# Autodesk Inventor assembly: IDLE ROLLER
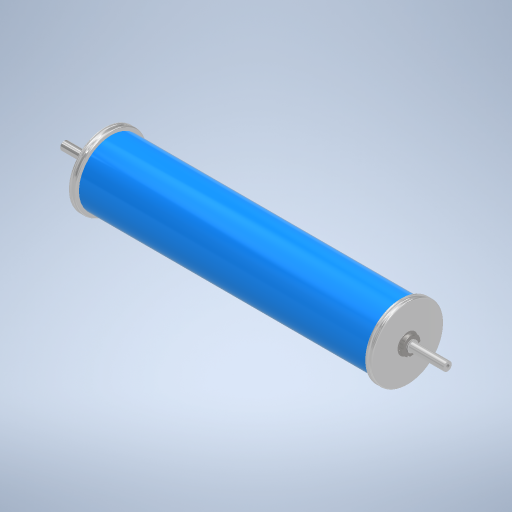
[picture p0: Inventor's stored thumbnail of the model, 512x512]
Saved by Autodesk Inventor 2023 (Build 270158000, 158)
## iProperties
Created: 2022-08-21
Part Number: IDLE ROLLER
Document SubType Name: Assembly
Designer: D.C. Eksteen
Mass: 1743.07 g
Surface Area: 2962.11 cm^2
Volume: 922.055 cm^3
Density: 1.89042 g/cm^3
Author: D.C. Eksteen
Title: FRONT ROLLER ASSEMBLY
## Documents named in this file (7)
- C:\Users\dylan\Desktop\Skripsie-2022\Design\CAD\IDLE ROLLER.iam
- C:\Users\dylan\Desktop\Skripsie\WORKSHOP\REMODELED\PARTS\BEARING.ipt
- C:\Users\dylan\Desktop\Skripsie\WORKSHOP\REMODELED\PARTS\LOCK NUT.ipt
- C:\Users\dylan\Desktop\Skripsie-2022\Design\CAD\IDLE ROLLER BAERING SPACER.ipt
- C:\Users\dylan\Desktop\Skripsie-2022\Design\CAD\IDLE ROLLER END CAP.ipt
- C:\Users\dylan\Desktop\Skripsie-2022\Design\CAD\IDLE ROLLER SHAFT.ipt
- C:\Users\dylan\Desktop\Skripsie-2022\Design\CAD\ROLLER TUBE.ipt
## Components (12 placed, 6 different names)
1. IDLE ROLLER END CAP:2
2. IDLE ROLLER END CAP:1
3. ROLLER TUBE:1
4. BS 290 SKF- with RS1 seal SKF 61902-RS1:3 — Mate:18
5. BS 290 SKF- with RS1 seal SKF 61902-RS1:2 — Mate:21
6. IDLE ROLLER SHAFT:1
7. ISO 2982-2 Locknuts(4 slots) M15 x 1 x 21:3 — Mate:16
8. ISO 2982-2 Locknuts(4 slots) M15 x 1 x 21:4 — Mate:23
9. BS 290 SKF- with RS1 seal SKF 61902-RS1:4 — Mate:16
10. IDLE ROLLER BAERING SPACER:1 — Mate:18
11. BS 290 SKF- with RS1 seal SKF 61902-RS1:5 — Mate:22, Mate:23
12. IDLE ROLLER BAERING SPACER:2 — Mate:21, Mate:22
## Relationships (23: Mate 22, Flush 1)
- [Mate]: IDLE ROLLER END CAP:1 ↔ ROLLER TUBE:1
- [Mate]: IDLE ROLLER END CAP:2 ↔ ROLLER TUBE:1
- [Mate]: IDLE ROLLER END CAP:1 ↔ ROLLER TUBE:1
- [Mate]: IDLE ROLLER END CAP:1 ↔ ROLLER TUBE:1
- [Mate]: IDLE ROLLER END CAP:2 ↔ ROLLER TUBE:1
- [Mate]: IDLE ROLLER END CAP:2 ↔ BS 290 SKF- with RS1 seal SKF 61902-RS1:3
- [Mate]: IDLE ROLLER END CAP:2 ↔ BS 290 SKF- with RS1 seal SKF 61902-RS1:3
- [Mate]: IDLE ROLLER END CAP:1 ↔ BS 290 SKF- with RS1 seal SKF 61902-RS1:2
- [Mate]: IDLE ROLLER END CAP:1 ↔ BS 290 SKF- with RS1 seal SKF 61902-RS1:2
- [Mate]: IDLE ROLLER END CAP:2 ↔ IDLE ROLLER SHAFT:1
- [Mate]: BS 290 SKF- with RS1 seal SKF 61902-RS1:3 ↔ IDLE ROLLER SHAFT:1
- [Mate]: IDLE ROLLER SHAFT:1 ↔ ISO 2982-2 Locknuts(4 slots) M15 x 1 x 21:3
- [Mate]: IDLE ROLLER SHAFT:1 ↔ ISO 2982-2 Locknuts(4 slots) M15 x 1 x 21:4
- [Mate]: IDLE ROLLER SHAFT:1 ↔ BS 290 SKF- with RS1 seal SKF 61902-RS1:4
- [Flush]: IDLE ROLLER END CAP:2 ↔ BS 290 SKF- with RS1 seal SKF 61902-RS1:4
- Mate:16: ISO 2982-2 Locknuts(4 slots) M15 x 1 x 21:3 ↔ BS 290 SKF- with RS1 seal SKF 61902-RS1:4
- [Mate]: IDLE ROLLER SHAFT:1 ↔ IDLE ROLLER BAERING SPACER:1
- Mate:18: BS 290 SKF- with RS1 seal SKF 61902-RS1:3 ↔ IDLE ROLLER BAERING SPACER:1
- [Mate]: IDLE ROLLER SHAFT:1 ↔ BS 290 SKF- with RS1 seal SKF 61902-RS1:5
- [Mate]: IDLE ROLLER SHAFT:1 ↔ IDLE ROLLER BAERING SPACER:2
- Mate:21: BS 290 SKF- with RS1 seal SKF 61902-RS1:2 ↔ IDLE ROLLER BAERING SPACER:2
- Mate:22: BS 290 SKF- with RS1 seal SKF 61902-RS1:5 ↔ IDLE ROLLER BAERING SPACER:2
- Mate:23: ISO 2982-2 Locknuts(4 slots) M15 x 1 x 21:4 ↔ BS 290 SKF- with RS1 seal SKF 61902-RS1:5
